# Autodesk Inventor assembly: MMCX_2DD-100P_Even
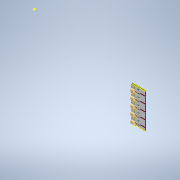
[picture p0: Inventor's stored thumbnail of the model, 180x180]
Saved by Autodesk Inventor 2020 (Build 240168000, 168)
## iProperties
Company: A Company
Created: 2019-09-04
Part Number: MMCX_2DD-100P_Even
Description: KiCad electronic assembly
Document SubType Name: Assembly
Designer: Eric
Authority: Unknown
Sending System: KiCad to STEP converter
Preprocessor: Open CASCADE STEP processor 6.9
Title: MMCX_2DD-100P_Even.step
Author: An Author
## Documents named in this file (3)
- C:\Users\Eric\OneDrive\KiCAD\MMCX_2DD-100P\MMCX_2DD-100P_Even.iam
- C:\Users\Eric\OneDrive\KiCAD\MMCX_2DD-100P\MMCX_Molex_73415-0961_Horizontal.iam
- C:\Users\Eric\OneDrive\KiCAD\MMCX_2DD-100P\SOLID_1_EVEN.ipt
## Components (11 placed, 11 different names)
1. 2 [sub-assembly] — Mate:1
2. 3 [sub-assembly]
3. 4 [sub-assembly]
4. 5 [sub-assembly]
5. 6 [sub-assembly]
6. 7 [sub-assembly]
7. 8 [sub-assembly]
8. 9 [sub-assembly]
9. 10 [sub-assembly]
10. 11 [sub-assembly]
11. 12 — Angle:1
## Relationships (2: Mate 1, Angle 1)
- Mate:1: 2
- Angle:1 (0 deg): 12
